# Autodesk Inventor assembly: PushrodRightNCS
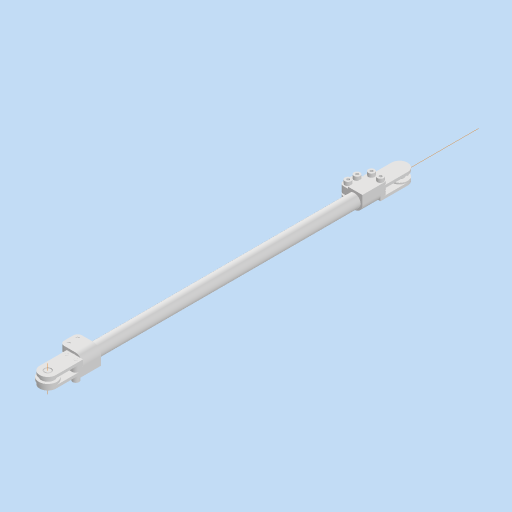
[picture p0: Inventor's stored thumbnail of the model, 512x512]
Saved by Autodesk Inventor 2023 (Build 270158000, 158)
## iProperties
Created: 2026-06-18
Part Number: PushrodRightNCS
Document SubType Name: Assembly
Designer: Nathann
Author: Nathann
## Documents named in this file (2)
- C:\Users\Nathann\ClawdDrive\Objet3D\RunningRobot\PartURDF\PushrodRightNCS.iam
- C:\Users\Nathann\ClawdDrive\Objet3D\RunningRobot\PartURDF\PushrodRight.iam
## Components (1 placed, 1 different names)
1. PushrodRight:1 [sub-assembly] — Mate:1, Flush:1, Mate:4
## Relationships (6: Mate 5, Flush 1)
- Mate:1: PushrodRight:1
- Mate:2
- Mate:3
- Flush:1: PushrodRight:1
- Mate:4: PushrodRight:1
- Mate:5
